# Autodesk Inventor assembly: Assembly
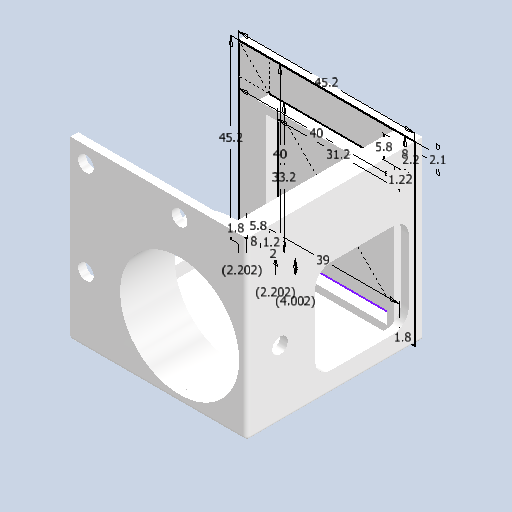
[picture p0: Inventor's stored thumbnail of the model, 512x512]
Saved by Autodesk Inventor 2023 (Build 270158000, 158)
## iProperties
Created: 2022-08-19
Part Number: Assembly
Document SubType Name: Assembly
Designer: Miner
Author: Miner
## Documents named in this file (3)
- D:\AKFS\OneDrive - RMIT University\0. Main Research\139. Spectral Camera\GiTHub\3D Design and Parts\Chamber assembly.iam
- D:\AKFS\OneDrive - RMIT University\0. Main Research\139. Spectral Camera\GiTHub\3D Design and Parts\Source files\Part02 Buttom cover.ipt
- D:\AKFS\OneDrive - RMIT University\0. Main Research\139. Spectral Camera\GiTHub\3D Design and Parts\Source files\Part01 Mirror chamber.ipt
## Components (2 placed, 2 different names)
1. Part02 Buttom cover:1 — Rigid:1
2. Part01 Mirror chamber:1 — Rigid:1
## Relationships (1: WeldJoint 1)
- Rigid:1 [WeldJoint]: Part02 Buttom cover:1 ↔ Part01 Mirror chamber:1
